# Autodesk Inventor assembly: Fixture Assembly
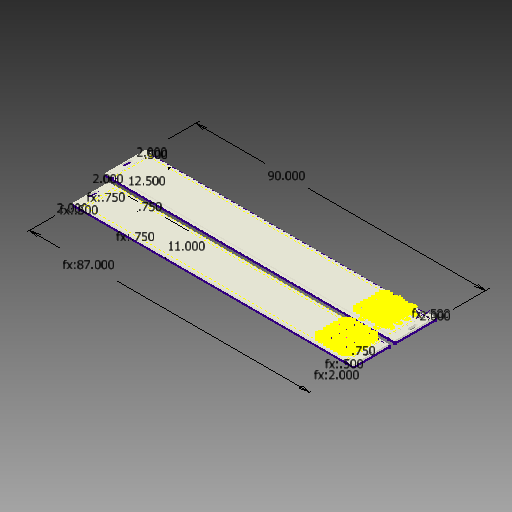
[picture p0: Inventor's stored thumbnail of the model, 512x512]
Saved by Autodesk Inventor 2018 (Build 220112000, 112)
## iProperties
Created: 2016-04-08
Part Number: Fixture Assembly
Document SubType Name: Assembly
Designer: Sam Clay
Author: Sam Clay
## Documents named in this file (6)
- Z:\enclosure\inventor\Fixture Assembly.iam
- Z:\enclosure\inventor\Fixture Base.ipt
- Z:\enclosure\inventor\Case Top Contour Fixture.ipt
- Z:\enclosure\inventor\Case Bottom Contour Fixture.ipt
- Z:\enclosure\inventor\Case Top Pocket Fixture.ipt
- Z:\enclosure\inventor\Case Bottom Pocket Fixture.ipt
## Components (33 placed, 5 different names)
1. Fixture Base:1 — Mate:27, Mate:28, Mate:35, Mate:36, Mate:38, Mate:40
2. Case Top Pocket Fixture:1 — Mate:34, Mate:35, Mate:36, Mate:39
3. Case Bottom Pocket Fixture:1 — Mate:34, Mate:38, Mate:39
4. Case Top Pocket Fixture:3
5. Case Bottom Pocket Fixture:2
6. Case Top Pocket Fixture:4
7. Case Bottom Pocket Fixture:3
8. Case Top Pocket Fixture:5
9. Case Bottom Pocket Fixture:4
10. Case Top Pocket Fixture:6
11. Case Bottom Pocket Fixture:5
12. Case Top Pocket Fixture:7
13. Case Bottom Pocket Fixture:6
14. Case Top Pocket Fixture:50
15. Case Bottom Pocket Fixture:49
16. Case Top Pocket Fixture:51
17. Case Bottom Pocket Fixture:50
18. Case Top Contour Fixture:1 — Mate:27, Mate:28, Mate:31, Mate:32, Mate:40
19. Case Bottom Contour Fixture:16 — Mate:31, Mate:32
20. Case Top Contour Fixture:2
21. Case Bottom Contour Fixture:17
22. Case Top Contour Fixture:3
23. Case Bottom Contour Fixture:18
24. Case Top Contour Fixture:4
25. Case Bottom Contour Fixture:19
26. Case Top Contour Fixture:5
27. Case Bottom Contour Fixture:20
28. Case Top Contour Fixture:6
29. Case Bottom Contour Fixture:21
30. Case Top Contour Fixture:7
31. Case Bottom Contour Fixture:22
32. Case Top Contour Fixture:8
33. Case Bottom Contour Fixture:23
## Component patterns: (1 elements), (1 elements), (8 elements, first: Case Top Pocket Fixture:1 + Case Bottom Pocket Fixture:1), (8 elements, first: Case Top Contour Fixture:1 + Case Bottom Contour Fixture:16)
## Relationships (10: Mate 10)
- Mate:27 (25.4 mm): Fixture Base:1 ↔ Case Top Contour Fixture:1
- Mate:28 (35.56 mm): Fixture Base:1 ↔ Case Top Contour Fixture:1
- Mate:31: Case Top Contour Fixture:1 ↔ Case Bottom Contour Fixture:16
- Mate:32 (7.8994 mm): Case Top Contour Fixture:1 ↔ Case Bottom Contour Fixture:16
- Mate:34: Case Top Pocket Fixture:1 ↔ Case Bottom Pocket Fixture:1
- Mate:35 (19.05 mm): Fixture Base:1 ↔ Case Top Pocket Fixture:1
- Mate:36 (3.175 mm): Fixture Base:1 ↔ Case Top Pocket Fixture:1
- Mate:38: Fixture Base:1 ↔ Case Bottom Pocket Fixture:1
- Mate:39 (7.8994 mm): Case Top Pocket Fixture:1 ↔ Case Bottom Pocket Fixture:1
- Mate:40 (17.78 mm): Fixture Base:1 ↔ Case Top Contour Fixture:1
